# Autodesk Inventor assembly: SSE2BSZ8-160
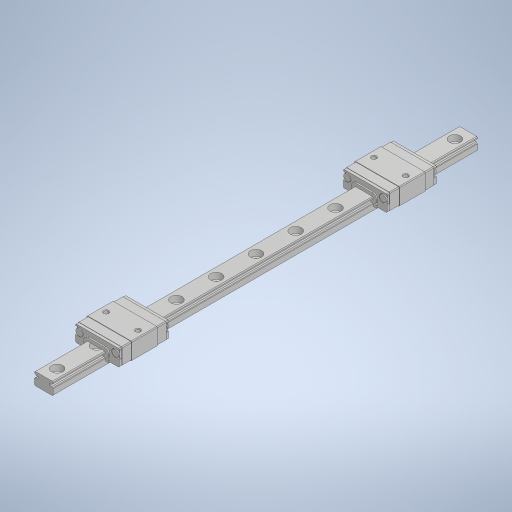
[picture p0: Inventor's stored thumbnail of the model, 512x512]
Saved by Autodesk Inventor 2024.3 (Build 283343010, 343A)
## iProperties
Company: CADENAS
Created: 2025-06-28
Part Number: SSE2BSZ8-160
Description: STEP AP203
Document SubType Name: Assembly
Designer: kshau
Sending System: PARTsolutions
Preprocessor: ST-DEVELOPER v19.3
Title: SSE2BSZ8-160
Author: License CC BY-ND 4.0
## Documents named in this file (3)
- C:\Users\kshau\Documents\inventor\Create_ViperX\NessesaryParts\SSE2BSZ8-160_STEP_AP203_20250628\SSE2BSZ8-160\SSE2BSZ8-160\SSE2BSZ8-160.iam
- C:\Users\kshau\Documents\inventor\Create_ViperX\NessesaryParts\SSE2BSZ8-160_STEP_AP203_20250628\SSE2BSZ8-160\SSE2BSZ8-160\SSE2BZ8-160_r1.ipt
- C:\Users\kshau\Documents\inventor\Create_ViperX\NessesaryParts\SSE2BSZ8-160_STEP_AP203_20250628\SSE2BSZ8-160\SSE2BSZ8-160\SEBSZ8_b.ipt
## Components (3 placed, 3 different names)
1. NAUO1 — スライダ:1, スライダ:2, フラッシュ:1, フラッシュ:2
2. NAUO2 — スライダ:1, フラッシュ:2
3. NAUO3 — スライダ:2, フラッシュ:1
## Relationships (4: TranslationJoint 2, Flush 2)
- スライダ:1 [TranslationJoint]: NAUO1 ↔ NAUO2
- スライダ:2 [TranslationJoint]: NAUO1 ↔ NAUO3
- フラッシュ:1 [Flush]: NAUO1 ↔ NAUO3
- フラッシュ:2 [Flush]: NAUO1 ↔ NAUO2
